# Autodesk Inventor assembly: flute
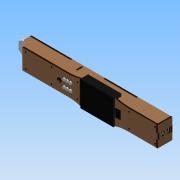
[picture p0: Inventor's stored thumbnail of the model, 180x180]
Saved by Autodesk Inventor 2015 (Build 190159000, 159)
## iProperties
Created: 2015-12-28
Part Number: flute
Document SubType Name: Assembly
Designer: Gregwar
Author: Gregwar
## Documents named in this file (10)
- C:\Users\Gregwar\Desktop\eFlute\3d\v1\flute.iam
- C:\Users\Gregwar\Desktop\eFlute\3d\v1\electronics.ipt
- C:\Users\Gregwar\Desktop\eFlute\3d\v1\bec.ipt
- C:\Users\Gregwar\Desktop\eFlute\3d\v1\top.ipt
- C:\Users\Gregwar\Desktop\eFlute\3d\v1\side.ipt
- C:\Users\Gregwar\Desktop\eFlute\3d\v1\bottom.ipt
- C:\Users\Gregwar\Desktop\eFlute\3d\v1\connectors.ipt
- C:\Users\Gregwar\Desktop\eFlute\3d\v1\bottom2.ipt
- C:\Users\Gregwar\Desktop\eFlute\3d\v1\button.ipt
- C:\Users\Gregwar\Desktop\eFlute\3d\v1\renfort.ipt
## Components (15 placed, 9 different names)
1. electronics:1 — Placage:1, Placage:2, Placage:3, Placage:19, Placage:20, Placage:21, Placage:22, Placage:23, Placage:24, Placage:25, Placage:26, Placage:27, Placage:28, Placage:29, Placage:30, Placage:38
2. bec:1 — Placage:1, Placage:2, Placage:3, Placage:4, Placage:5, Placage:6, Placage:10, Placage:11, Placage:36
3. top:1 — Placage:4, Placage:5, Placage:6, Placage:7, Affleurement:1, Affleurement:2, Placage:8, Affleurement:3, Affleurement:4, Placage:14, Affleurement:6, Placage:36, Placage:38, Placage:39
4. side:1 — Placage:7, Affleurement:1, Affleurement:2, Affleurement:7, Affleurement:14, Placage:40
5. side:2 — Placage:8, Affleurement:3, Affleurement:4, Placage:9, Placage:15, Affleurement:9, Placage:37
6. bottom:1 — Placage:9, Placage:10, Placage:11, Placage:37
7. connectors:1 — Placage:14, Affleurement:6, Affleurement:7, Affleurement:8, Affleurement:13
8. bottom2:1 — Placage:15, Affleurement:8, Affleurement:9, Affleurement:13
9. button:1 — Placage:19, Placage:20
10. button:2 — Placage:21, Placage:22
11. button:3 — Placage:23, Placage:24
12. button:4 — Placage:25, Placage:26
13. button:5 — Placage:27, Placage:28
14. button:6 — Placage:29, Placage:30
15. renfort:3 — Placage:39, Affleurement:14, Placage:40
## Relationships (40: Mate 30, Flush 10)
- Placage:1 [Mate]: electronics:1 ↔ bec:1
- Placage:2 [Mate]: electronics:1 ↔ bec:1
- Placage:3 [Mate]: electronics:1 ↔ bec:1
- Placage:4 [Mate]: bec:1 ↔ top:1
- Placage:5 [Mate]: bec:1 ↔ top:1
- Placage:6 [Mate]: bec:1 ↔ top:1
- Placage:7 [Mate]: top:1 ↔ side:1
- Affleurement:1 [Flush]: top:1 ↔ side:1
- Affleurement:2 [Flush]: top:1 ↔ side:1
- Placage:8 [Mate]: top:1 ↔ side:2
- Affleurement:3 [Flush]: top:1 ↔ side:2
- Affleurement:4 [Flush]: top:1 ↔ side:2
- Placage:9 [Mate]: side:2 ↔ bottom:1
- Placage:10 [Mate]: bec:1 ↔ bottom:1
- Placage:11 [Mate]: bec:1 ↔ bottom:1
- Placage:14 [Mate]: top:1 ↔ connectors:1
- Affleurement:6 [Flush]: top:1 ↔ connectors:1
- Affleurement:7 [Flush]: side:1 ↔ connectors:1
- Placage:15 [Mate]: side:2 ↔ bottom2:1
- Affleurement:8 [Flush]: connectors:1 ↔ bottom2:1
- Affleurement:9 [Flush]: side:2 ↔ bottom2:1
- Placage:19 [Mate]: electronics:1 ↔ button:1
- Placage:20 [Mate]: electronics:1 ↔ button:1
- Placage:21 [Mate]: electronics:1 ↔ button:2
- Placage:22 [Mate]: electronics:1 ↔ button:2
- Placage:23 [Mate]: electronics:1 ↔ button:3
- Placage:24 [Mate]: electronics:1 ↔ button:3
- Placage:25 [Mate]: electronics:1 ↔ button:4
- Placage:26 [Mate]: electronics:1 ↔ button:4
- Placage:27 [Mate]: electronics:1 ↔ button:5
- Placage:28 [Mate]: electronics:1 ↔ button:5
- Placage:29 [Mate]: electronics:1 ↔ button:6
- Placage:30 [Mate]: electronics:1 ↔ button:6
- Placage:36 [Mate]: bec:1 ↔ top:1
- Placage:37 [Mate]: side:2 ↔ bottom:1
- Placage:38 [Mate] (0.5 mm): electronics:1 ↔ top:1
- Affleurement:13 [Flush]: connectors:1 ↔ bottom2:1
- Placage:39 [Mate]: top:1 ↔ renfort:3
- Affleurement:14 [Flush]: side:1 ↔ renfort:3
- Placage:40 [Mate]: side:1 ↔ renfort:3
